# Autodesk Inventor assembly: ASY дренаж угольные
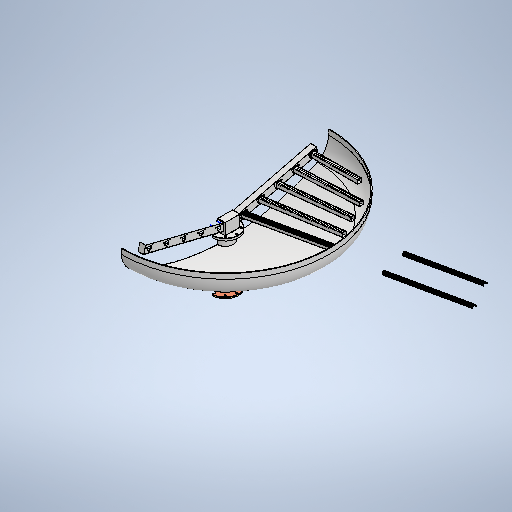
[picture p0: Inventor's stored thumbnail of the model, 512x512]
Saved by Autodesk Inventor 2025 (Build 290162010, 162A)
## iProperties
Created: 2024-12-09
Part Number: ASY дренаж угольные
Document SubType Name: Assembly
Designer: user
Author: user
## Documents named in this file (24)
- C:\Users\admin\YandexDisk-badmisterfox\home pc\Inventor\Manturovo\Manturovo_Se-clar\Дренаж на угольные\ASY дренаж угольные.iam
- C:\Users\admin\YandexDisk-badmisterfox\home pc\Inventor\Manturovo\Manturovo_Se-clar\Дренаж на угольные\Main filter Flange.ipt
- C:\Users\admin\YandexDisk-badmisterfox\home pc\Inventor\Manturovo\Manturovo_Se-clar\Дренаж на угольные\drain flange.ipt
- C:\Users\admin\YandexDisk-badmisterfox\home pc\Inventor\Manturovo\Manturovo_Se-clar\Дренаж на угольные\Part9.ipt
- C:\Users\admin\YandexDisk-badmisterfox\home pc\Inventor\Manturovo\Manturovo_Se-clar\Дренаж на угольные\drain bottom plate.ipt
- C:\Users\admin\YandexDisk-badmisterfox\home pc\Inventor\Manturovo\Manturovo_Se-clar\Дренаж на угольные\drain wall with flange.ipt
- C:\Users\admin\YandexDisk-badmisterfox\home pc\Inventor\Manturovo\Content Center Files\en-US\DIN 933\DIN 933 - M12  x 35.ipt
- C:\Users\admin\YandexDisk-badmisterfox\home pc\Inventor\Manturovo\Manturovo_Se-clar\Дренаж на угольные\drain cup.ipt
- C:\Users\admin\YandexDisk-badmisterfox\home pc\Inventor\Manturovo\Manturovo_Se-clar\Дренаж на угольные\Фильтр напорный угольный 30 куб час.ipt
- C:\Users\admin\YandexDisk-badmisterfox\home pc\Inventor\Manturovo\Manturovo_Se-clar\Дренаж на угольные\MNT-CDF-401 roof 1.ipt
- C:\Users\admin\YandexDisk-badmisterfox\home pc\Inventor\Manturovo\Manturovo_Se-clar\Дренаж на угольные\MNT-CDF-501 box.ipt
- C:\Users\admin\YandexDisk-badmisterfox\home pc\Inventor\Manturovo\Manturovo_Se-clar\Дренаж на угольные\MNT-CDF-502 tube.ipt
- C:\Users\admin\YandexDisk-badmisterfox\home pc\Inventor\Manturovo\Manturovo_Se-clar\Дренаж на угольные\MNT-CDF-503  main tube 1.ipt
- C:\Users\admin\YandexDisk-badmisterfox\home pc\Inventor\Manturovo\Content Center Files\en-US\DIN 933\DIN 933 - M8  x 20.ipt
- C:\Users\admin\YandexDisk-badmisterfox\home pc\Inventor\Manturovo\Manturovo_Se-clar\Дренаж на угольные\MNT-CDF-504 small tube flange.ipt
- C:\Users\admin\YandexDisk-badmisterfox\home pc\Inventor\Manturovo\Manturovo_Se-clar\Дренаж на угольные\MNT-CDF-315 beam 5.ipt
- C:\Users\admin\YandexDisk-badmisterfox\home pc\Inventor\Manturovo\Manturovo_Se-clar\Дренаж на угольные\MNT-CDF-312 beam 2.ipt
- C:\Users\admin\YandexDisk-badmisterfox\home pc\Inventor\Manturovo\Manturovo_Se-clar\Дренаж на угольные\MNT-CDF-313 beam 3.ipt
- C:\Users\admin\YandexDisk-badmisterfox\home pc\Inventor\Manturovo\Manturovo_Se-clar\Дренаж на угольные\MNT-CDF-314 beam 4.ipt
- C:\Users\admin\YandexDisk-badmisterfox\home pc\Inventor\Manturovo\Manturovo_Se-clar\Дренаж на угольные\MNT-CDF-601 CAP.ipt
- C:\Users\admin\YandexDisk-badmisterfox\home pc\Inventor\Manturovo\Manturovo_Se-clar\Дренаж на угольные\MNT-CDF-602 CAP.ipt
- C:\Users\admin\YandexDisk-badmisterfox\home pc\Inventor\Manturovo\Manturovo_Se-clar\Дренаж на угольные\MNT-CDF-603 CAP.ipt
- C:\Users\admin\YandexDisk-badmisterfox\home pc\Inventor\Manturovo\Manturovo_Se-clar\Дренаж на угольные\ASY Луч 1.iam
- C:\Users\admin\YandexDisk-badmisterfox\home pc\Inventor\Manturovo\Manturovo_Se-clar\Дренаж на угольные\MNT-CDF-402 roof 2.ipt
## Components (43 placed, 23 different names)
1. Main filter Flange.ipt:1 — Rigid:1
2. drain flange.ipt:1 — Rigid:1, Rigid:7
3. Part9.ipt:1 — Rigid:4, Rigid:7
4. drain bottom plate.ipt:1 — Rigid:4, Rigid:5, Rigid:6
5. drain wall with flange:1 — Rigid:3, Rigid:6, Mate:2, Flush:1, Rotational:2, Rotational:3, Rotational:4
6. DIN 933 - replaced by DIN EN 24017 M12  x 35:1 — Rigid:3
7. drain wall with flange:2 — Rigid:5, Mate:1, Rotational:1
8. DIN 933 - replaced by DIN EN 24017 M12  x 35:2 — Rotational:1
9. DIN 933 - replaced by DIN EN 24017 M12  x 35:3 — Rotational:3
10. Part1:3 — Mate:1, Mate:2, Flush:1, Rotational:5, Rotational:6
11. DIN 933 - replaced by DIN EN 24017 M12  x 35:4 — Rotational:2
12. DIN 933 - replaced by DIN EN 24017 M12  x 35:5 — Rotational:4
13. DIN 933 - replaced by DIN EN 24017 M12  x 35:6 — Rotational:6
14. DIN 933 - replaced by DIN EN 24017 M12  x 35:7 — Rotational:5
15. Фильтр напорный угольный 30 куб час:1 — Mate:4, Flush:3, Flush:4, Rigid:12
16. MNT-CDF-501 box:1 — Rotational:9, Flush:8, Mate:9, Mate:10, Rotational:10, Rotational:11, Rigid:32, Rigid:34
17. drain flange:2 — Rigid:12, Mate:5
18. MNT-CDF-502 tube:4 — Rotational:11
19. MNT-CDF-502 tube:3 — Rotational:10
20. MNT-CDF-502 tube:2 — Rotational:9
21. MNT-CDF-503  main tube 1:1 — Rigid:14, Rigid:15
22. MNT-CDF-503  main tube 1:2 — Rigid:14, Mate:5, Mate:6, Mate:9, Mate:10, Rigid:29
23. MNT-CDF-501 box:2 — Rigid:15, Rigid:19, Rigid:20, Rigid:23, Rigid:24, Rigid:25, Rigid:33, Rigid:35
24. DIN 933 - replaced by DIN EN 24017 M8  x 20:1
25. MNT-CDF-502 tube:5 — Rigid:19
26. MNT-CDF-315 beam 5:1 — Rigid:21
27. Part1:5 — Rigid:20, Rigid:21
28. DIN 933 - replaced by DIN EN 24017 M8  x 20:2
29. DIN 933 - replaced by DIN EN 24017 M8  x 20:3
30. MNT-CDF-312 beam 2:1 — Rigid:26
31. Part1:6 — Rigid:23, Rigid:26
32. Part1:7 — Rigid:24, Rigid:27
33. Part1:8 — Rigid:25, Rigid:28
34. MNT-CDF-313 beam 3:1 — Rigid:27
35. MNT-CDF-314 beam 4:1 — Rigid:28
36. MNT-CDF-601 CAP:1 — Rigid:29
37. MNT-CDF-602 CAP:1 — Rigid:32
38. MNT-CDF-602 CAP:2 — Rigid:33
39. MNT-CDF-603 CAP:1 — Rigid:34
40. MNT-CDF-603 CAP:2 — Rigid:35
41. ASY Луч 1:1 [sub-assembly]
42. MNT-CDF-401 roof 1:1
43. MNT-CDF-402 roof 2:1
## Relationships (47: WeldJoint 24, RevoluteJoint 12, Mate 7, Flush 4)
- Rigid:1 [WeldJoint]: Main filter Flange.ipt:1 ↔ drain flange.ipt:1
- Rigid:3 [WeldJoint]: drain wall with flange:1 ↔ DIN 933 - replaced by DIN EN 24017 M12  x 35:1
- Rigid:4 [WeldJoint]: Part9.ipt:1 ↔ drain bottom plate.ipt:1
- Rigid:5 [WeldJoint]: drain bottom plate.ipt:1 ↔ drain wall with flange:2
- Rigid:6 [WeldJoint]: drain bottom plate.ipt:1 ↔ drain wall with flange:1
- Rotational:1 [RevoluteJoint]: drain wall with flange:2 ↔ DIN 933 - replaced by DIN EN 24017 M12  x 35:2
- Rigid:7 [WeldJoint]: drain flange.ipt:1 ↔ Part9.ipt:1
- Mate:1: drain wall with flange:2 ↔ Part1:3
- Mate:2: drain wall with flange:1 ↔ Part1:3
- Flush:1: drain wall with flange:1 ↔ Part1:3
- Rotational:2 [RevoluteJoint]: drain wall with flange:1 ↔ DIN 933 - replaced by DIN EN 24017 M12  x 35:4
- Rotational:3 [RevoluteJoint]: drain wall with flange:1 ↔ DIN 933 - replaced by DIN EN 24017 M12  x 35:3
- Rotational:4 [RevoluteJoint]: drain wall with flange:1 ↔ DIN 933 - replaced by DIN EN 24017 M12  x 35:5
- Rotational:5 [RevoluteJoint]: Part1:3 ↔ DIN 933 - replaced by DIN EN 24017 M12  x 35:7
- Rotational:6 [RevoluteJoint]: Part1:3 ↔ DIN 933 - replaced by DIN EN 24017 M12  x 35:6
- Mate:4: Фильтр напорный угольный 30 куб час:1
- Flush:3: Фильтр напорный угольный 30 куб час:1
- Flush:4: Фильтр напорный угольный 30 куб час:1
- Rigid:12 [WeldJoint]: Фильтр напорный угольный 30 куб час:1 ↔ drain flange:2
- Rotational:9 [RevoluteJoint]: MNT-CDF-501 box:1 ↔ MNT-CDF-502 tube:2
- Rigid:14 [WeldJoint]: MNT-CDF-503  main tube 1:1 ↔ MNT-CDF-503  main tube 1:2
- Mate:5: drain flange:2 ↔ MNT-CDF-503  main tube 1:2
- Mate:6: MNT-CDF-503  main tube 1:2
- Flush:8: MNT-CDF-501 box:1
- Mate:9: MNT-CDF-501 box:1 ↔ MNT-CDF-503  main tube 1:2
- Mate:10: MNT-CDF-501 box:1 ↔ MNT-CDF-503  main tube 1:2
- Rigid:15 [WeldJoint]: MNT-CDF-503  main tube 1:1 ↔ MNT-CDF-501 box:2
- Rotational:10 [RevoluteJoint]: MNT-CDF-501 box:1 ↔ MNT-CDF-502 tube:3
- Rotational:11 [RevoluteJoint]: MNT-CDF-501 box:1 ↔ MNT-CDF-502 tube:4
- [WeldJoint]: MNT-CDF-501 box:2 ↔ ASY Луч 1:1
- Rigid:19 [WeldJoint]: MNT-CDF-501 box:2 ↔ MNT-CDF-502 tube:5
- Rigid:20 [WeldJoint]: MNT-CDF-501 box:2 ↔ Part1:5
- Rigid:21 [WeldJoint]: MNT-CDF-315 beam 5:1 ↔ Part1:5
- Rigid:23 [WeldJoint]: MNT-CDF-501 box:2 ↔ Part1:6
- Rigid:24 [WeldJoint]: MNT-CDF-501 box:2 ↔ Part1:7
- Rigid:25 [WeldJoint]: MNT-CDF-501 box:2 ↔ Part1:8
- Rigid:26 [WeldJoint]: MNT-CDF-312 beam 2:1 ↔ Part1:6
- Rigid:27 [WeldJoint]: Part1:7 ↔ MNT-CDF-313 beam 3:1
- Rigid:28 [WeldJoint]: Part1:8 ↔ MNT-CDF-314 beam 4:1
- Rigid:29 [WeldJoint]: MNT-CDF-503  main tube 1:2 ↔ MNT-CDF-601 CAP:1
- Rigid:32 [WeldJoint]: MNT-CDF-501 box:1 ↔ MNT-CDF-602 CAP:1
- Rigid:33 [WeldJoint]: MNT-CDF-501 box:2 ↔ MNT-CDF-602 CAP:2
- Rigid:34 [WeldJoint]: MNT-CDF-501 box:1 ↔ MNT-CDF-603 CAP:1
- Rigid:35 [WeldJoint]: MNT-CDF-501 box:2 ↔ MNT-CDF-603 CAP:2
- [RevoluteJoint]: DIN 933 - replaced by DIN EN 24017 M8  x 20:2 ↔ ASY Луч 1:1
- [RevoluteJoint]: DIN 933 - replaced by DIN EN 24017 M8  x 20:3 ↔ ASY Луч 1:1
- [RevoluteJoint]: DIN 933 - replaced by DIN EN 24017 M8  x 20:1 ↔ ASY Луч 1:1
